# Autodesk Inventor assembly: PistonV2
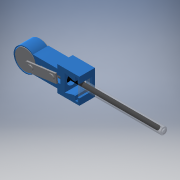
[picture p0: Inventor's stored thumbnail of the model, 180x180]
Saved by Autodesk Inventor 2016 (Build 200138000, 138)
## iProperties
Created: 2017-03-04
Part Number: PistonV2
Document SubType Name: Assembly
Designer: Owner
Author: Owner
## Documents named in this file (11)
- C:\Users\Owner\Documents\Inventor\TSA\2017\Animatronics\Alligator\Pistons\PistonHead\PistonV2.iam
- C:\Users\Owner\Documents\Inventor\TSA\2017\Animatronics\Alligator\Pistons\PistonHead\PistonV2.ipt
- C:\Users\Owner\Documents\Inventor\TSA\2017\Animatronics\Alligator\Pistons\PistonHead\PistonCylinder.ipt
- C:\Users\Owner\Documents\Inventor\TSA\2017\Animatronics\Alligator\Pistons\PistonHead\RotationDisk.ipt
- C:\Users\Owner\Documents\Inventor\TSA\2017\Animatronics\Alligator\Pistons\PistonHead\Sealer.ipt
- C:\Users\Owner\Documents\Inventor\TSA\2017\Animatronics\Alligator\Pistons\Syringe1mL\SyringeBody.ipt
- C:\Users\Owner\Documents\Inventor\TSA\2017\Animatronics\Alligator\Pistons\Syringe1mL\SyringEnd.ipt
- C:\Users\Owner\Documents\Inventor\TSA\2017\Animatronics\Alligator\Pistons\PistonHead\PinLarge.ipt
- C:\Users\Owner\Documents\Inventor\TSA\2017\Animatronics\Alligator\Pistons\PistonHead\PinSmall.ipt
- C:\Users\Owner\Documents\Inventor\TSA\2017\Animatronics\Alligator\Pistons\PistonHead\Connector.ipt
- C:\Users\Owner\Documents\Inventor\TSA\2017\Animatronics\Alligator\Mock Parts\servo (2).ipt
## Components (10 placed, 10 different names)
1. PistonV2:1 — Mate:2, Flush:2, Mate:3, Mate:5, Mate:7, Angle:1, Mate:8, Angle:2, Mate:16, Angle:3
2. PistonCylinder:1 — Mate:8, Mate:9, Mate:10, Mate:11
3. RotationDisk:1 — Mate:2, Flush:2, Mate:4, Flush:4, Mate:13
4. Sealer:1 — Mate:3, Mate:4, Mate:15
5. SyringeBody:1 — Mate:6, Mate:7, Angle:1
6. SyringEnd:1 — Mate:5, Mate:6, Mate:9
7. PinLarge:1 — Mate:10, Mate:11, Angle:2, Mate:12
8. PinSmall:1 — Mate:13, Mate:14
9. Connector:1 — Flush:4, Mate:12, Mate:14
10. servo (2):1 — Mate:15, Mate:16, Angle:3
## Relationships (20: Mate 15, Angle 3, Flush 2)
- Mate:2: PistonV2:1 ↔ RotationDisk:1
- Flush:2: PistonV2:1 ↔ RotationDisk:1
- Mate:3: PistonV2:1 ↔ Sealer:1
- Mate:4: RotationDisk:1 ↔ Sealer:1
- Mate:5: PistonV2:1 ↔ SyringEnd:1
- Mate:6: SyringeBody:1 ↔ SyringEnd:1
- Mate:7 (0.25 mm): PistonV2:1 ↔ SyringeBody:1
- Angle:1 (0 deg): PistonV2:1 ↔ SyringeBody:1
- Mate:8: PistonV2:1 ↔ PistonCylinder:1
- Mate:9: PistonCylinder:1 ↔ SyringEnd:1
- Mate:10: PistonCylinder:1 ↔ PinLarge:1
- Mate:11: PistonCylinder:1 ↔ PinLarge:1
- Angle:2 (0 deg): PistonV2:1 ↔ PinLarge:1
- Flush:4: RotationDisk:1 ↔ Connector:1
- Mate:12: PinLarge:1 ↔ Connector:1
- Mate:13: RotationDisk:1 ↔ PinSmall:1
- Mate:14: PinSmall:1 ↔ Connector:1
- Mate:15: Sealer:1 ↔ servo (2):1
- Mate:16: PistonV2:1 ↔ servo (2):1
- Angle:3 (0 deg): PistonV2:1 ↔ servo (2):1
